# Autodesk Inventor assembly: The Claw
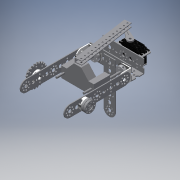
[picture p0: Inventor's stored thumbnail of the model, 180x180]
Saved by Autodesk Inventor 2019 (Build 230136000, 136)
## iProperties
Created: 2019-11-23
Part Number: The Claw
Document SubType Name: Assembly
Designer: User
Author: User
## Documents named in this file (15)
- C:\Robotics\CAD\2019-20_CAD\Collection\The Claw.iam
- C:\Robotics\CAD\2019-20_CAD\Collection\sliding piece for grabber.ipt
- C:\Robotics\CAD\COTSParts\Tetrix\Tetrix Flat bar 160 mm.ipt
- C:\Robotics\CAD\COTSParts\Tetrix\Tetrix shaft 100mm.ipt
- C:\Robotics\CAD\COTSParts\Tetrix\Tetrix Hub - axle_MIR.ipt
- C:\Robotics\CAD\2019-20_CAD\Collection\Cut bar with grip.ipt
- C:\Robotics\CAD\2019-20_CAD\Collection\Cut piece for bar.ipt
- C:\Robotics\CAD\COTSParts\Tetrix\Tetrix bracket - angle.ipt
- C:\Robotics\CAD\COTSParts\Tetrix\Tetrix bracket - single servo.ipt
- C:\Robotics\CAD\COTSParts\Tetrix\Tetrix 180 Servo.ipt
- C:\Robotics\CAD\COTSParts\Actobotics\545 parts\545364 assembly.ipt
- C:\Robotics\CAD\COTSParts\Actobotics\545 parts\545456PatternAdapter.77in.625in.ipt
- C:\Robotics\CAD\COTSParts\Sprockets - AndyMark\615106.ipt
- C:\Robotics\CAD\2019-20_CAD\Collection\Servo Bar.ipt
- C:\Robotics\CAD\2019-20_CAD\Collection\Servo horn.ipt
## Components (20 placed, 14 different names)
1. Tetrix Flat bar 160 mm:1 — Mate:19, Mate:20, Angle:5, Mate:30, Mate:31
2. Tetrix Flat bar 160 mm:2 — Mate:17, Mate:18, Angle:4, Mate:25, Mate:26
3. Tetrix shaft 100mm:1 — Flush:1, Mate:3, Mate:9
4. Tetrix shaft 100mm:2 — Flush:1, Mate:4, Mate:8, Flush:3
5. Tetrix Hub - axle_MIR:1 — Mate:3, Flush:2, Mate:7, Mate:16
6. Tetrix Hub - axle_MIR:2 — Mate:4, Flush:2, Mate:6
7. Cut bar with grip:1 — Mate:10, Mate:11, Angle:1
8. Cut piece for bar:1 — Mate:6, Mate:7, Mate:10, Mate:11, Angle:1, Mate:12, Mate:13, Angle:2, Mate:14, Mate:15, Angle:3, Mate:21, Mate:22, Angle:6, Flush:3
9. sliding piece for grabber:1 — Mate:8, Mate:9, Mate:40, Mate:41
10. Tetrix bracket - angle:1 — Mate:12, Mate:13, Angle:2, Mate:17, Mate:18, Angle:4
11. Tetrix bracket - angle:2 — Mate:14, Mate:15, Angle:3, Mate:16, Mate:19, Mate:20, Angle:5
12. Tetrix bracket - single servo:1 — Mate:21, Mate:22, Angle:6, Mate:23, Mate:24, Angle:7
13. Tetrix 180 Servo:1 — Mate:23, Mate:24, Angle:7, Mate:38, Mate:39
14. 545364 assembly:1 — Mate:35, Mate:36, Mate:37
15. 545364 assembly:2 — Mate:27, Mate:28, Mate:29
16. 545456PatternAdapter.77in.625in:1 — Mate:30, Mate:31, Mate:32, Mate:33, Mate:34, Mate:37
17. 545456PatternAdapter.77in.625in:2 — Mate:25, Mate:26, Mate:27, Mate:28, Mate:29
18. 615106:1 — Mate:32, Mate:33, Mate:34, Mate:35, Mate:36
19. Servo Bar:1 — Mate:40, Mate:41, Mate:42
20. Servo horn:1 — Mate:38, Mate:39, Mate:42
## Relationships (49: Mate 39, Angle 7, Flush 3)
- Flush:1: Tetrix shaft 100mm:1 ↔ Tetrix shaft 100mm:2
- Mate:3: Tetrix shaft 100mm:1 ↔ Tetrix Hub - axle_MIR:1
- Mate:4: Tetrix shaft 100mm:2 ↔ Tetrix Hub - axle_MIR:2
- Flush:2: Tetrix Hub - axle_MIR:1 ↔ Tetrix Hub - axle_MIR:2
- Mate:6: Tetrix Hub - axle_MIR:2 ↔ Cut piece for bar:1
- Mate:7 (0.508 mm): Tetrix Hub - axle_MIR:1 ↔ Cut piece for bar:1
- Mate:8: Tetrix shaft 100mm:2 ↔ sliding piece for grabber:1
- Mate:9: Tetrix shaft 100mm:1 ↔ sliding piece for grabber:1
- Mate:10: Cut bar with grip:1 ↔ Cut piece for bar:1
- Mate:11: Cut bar with grip:1 ↔ Cut piece for bar:1
- Angle:1 (0 deg): Cut bar with grip:1 ↔ Cut piece for bar:1
- Mate:12: Cut piece for bar:1 ↔ Tetrix bracket - angle:1
- Mate:13: Cut piece for bar:1 ↔ Tetrix bracket - angle:1
- Angle:2 (0 deg): Cut piece for bar:1 ↔ Tetrix bracket - angle:1
- Mate:14: Cut piece for bar:1 ↔ Tetrix bracket - angle:2
- Mate:15: Cut piece for bar:1 ↔ Tetrix bracket - angle:2
- Angle:3 (0 deg): Cut piece for bar:1 ↔ Tetrix bracket - angle:2
- Mate:16: Tetrix Hub - axle_MIR:1 ↔ Tetrix bracket - angle:2
- Mate:17: Tetrix Flat bar 160 mm:2 ↔ Tetrix bracket - angle:1
- Mate:18: Tetrix Flat bar 160 mm:2 ↔ Tetrix bracket - angle:1
- Angle:4 (0 deg): Tetrix Flat bar 160 mm:2 ↔ Tetrix bracket - angle:1
- Mate:19: Tetrix Flat bar 160 mm:1 ↔ Tetrix bracket - angle:2
- Mate:20: Tetrix Flat bar 160 mm:1 ↔ Tetrix bracket - angle:2
- Angle:5 (0 deg): Tetrix Flat bar 160 mm:1 ↔ Tetrix bracket - angle:2
- Mate:21: Cut piece for bar:1 ↔ Tetrix bracket - single servo:1
- Mate:22: Cut piece for bar:1 ↔ Tetrix bracket - single servo:1
- Angle:6 (0 deg): Cut piece for bar:1 ↔ Tetrix bracket - single servo:1
- Mate:23: Tetrix bracket - single servo:1 ↔ Tetrix 180 Servo:1
- Mate:24: Tetrix bracket - single servo:1 ↔ Tetrix 180 Servo:1
- Angle:7 (180 deg): Tetrix bracket - single servo:1 ↔ Tetrix 180 Servo:1
- Mate:25: Tetrix Flat bar 160 mm:2 ↔ 545456PatternAdapter.77in.625in:2
- Mate:26: Tetrix Flat bar 160 mm:2 ↔ 545456PatternAdapter.77in.625in:2
- Mate:27: 545364 assembly:2 ↔ 545456PatternAdapter.77in.625in:2
- Mate:28: 545364 assembly:2 ↔ 545456PatternAdapter.77in.625in:2
- Mate:29: 545364 assembly:2 ↔ 545456PatternAdapter.77in.625in:2
- Mate:30: Tetrix Flat bar 160 mm:1 ↔ 545456PatternAdapter.77in.625in:1
- Mate:31: Tetrix Flat bar 160 mm:1 ↔ 545456PatternAdapter.77in.625in:1
- Mate:32: 545456PatternAdapter.77in.625in:1 ↔ 615106:1
- Mate:33: 545456PatternAdapter.77in.625in:1 ↔ 615106:1
- Mate:34: 545456PatternAdapter.77in.625in:1 ↔ 615106:1
- Mate:35: 545364 assembly:1 ↔ 615106:1
- Mate:36: 545364 assembly:1 ↔ 615106:1
- Mate:37: 545364 assembly:1 ↔ 545456PatternAdapter.77in.625in:1
- Mate:38: Tetrix 180 Servo:1 ↔ Servo horn:1
- Mate:39: Tetrix 180 Servo:1 ↔ Servo horn:1
- Mate:40: sliding piece for grabber:1 ↔ Servo Bar:1
- Mate:41: sliding piece for grabber:1 ↔ Servo Bar:1
- Flush:3 (3.6576 mm): Tetrix shaft 100mm:2 ↔ Cut piece for bar:1
- Mate:42: Servo Bar:1 ↔ Servo horn:1
